# Autodesk Inventor assembly: Tetrix_739083
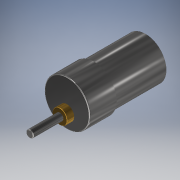
[picture p0: Inventor's stored thumbnail of the model, 180x180]
Saved by Autodesk Inventor 2019 (Build 230136000, 136)
## iProperties
Category: Motors
Company: Autodesk Inc.
Created: 2014-11-19
Part Number: Tetrix_739083
Document SubType Name: Assembly
Designer: Tetrix
Catalog Web Link: http://www.tetrixrobotics.com/TETRIX_DC_Gear_Motor
Vendor: Tetrix
Author: Autodesk Inc.
## Documents named in this file (3)
- C:\Users\tbloo\Documents\Inventor\FTC Tetrix KOP\Miscellaneous\Tetrix_39083.iam
- C:\Users\tbloo\Downloads\FTC Tetrix KOP\Miscellaneous\Tetrix_39083_Motor.ipt
- C:\Users\tbloo\Downloads\FTC Tetrix KOP\Miscellaneous\Tetrix_39083_Axle.ipt
## Components (2 placed, 2 different names)
1. Tetrix_739083_Motor — Insert:1
2. Tetrix_739083_Axle — Insert:1
## Relationships (1: Insert 1)
- Insert:1: Tetrix_739083_Motor ↔ Tetrix_739083_Axle
